# Autodesk Inventor assembly: Ramps 1.4
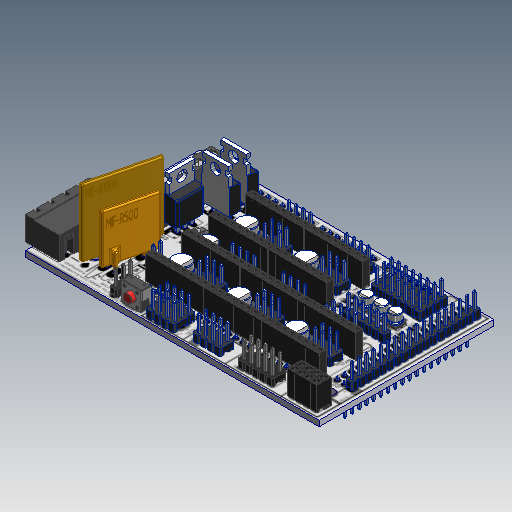
[picture p0: Inventor's stored thumbnail of the model, 512x512]
Saved by Autodesk Inventor 2017 (Build 210142000, 142)
## iProperties
Created: 2012-11-13
Part Number: Ramps 1.4
Document SubType Name: Ensemble
Mass: 53.1508 g
Surface Area: 690.991 cm^2
Volume: 42.1194 cm^3
Density: 1.26191 g/cm^3
Stock Number: 1420-11-20
Sending System: SolidWorks 2013
Preprocessor: SwSTEP 2.0
Title: RAMPS1_4.STEP
## Documents named in this file (24)
- W:\Professionnel\Conception FABLAB\1420-Vauban 3D XL\1420-11 Electronique\1420-11-20 Ramps\1420-11-20 Ramps 1.4.iam
- W:\Professionnel\Conception FABLAB\1420-Vauban 3D XL\1420-11 Electronique\1420-11-20 Ramps\RAMPS1_4.ipt
- W:\Professionnel\Conception FABLAB\1420-Vauban 3D XL\1420-11 Electronique\1420-11-20 Ramps\User Library-POWER MOSFET, NON-SURFACE-MOUNT.ipt
- W:\Professionnel\Conception FABLAB\1420-Vauban 3D XL\1420-11 Electronique\1420-11-20 Ramps\female_header_a-bl254-dg-g08d.ipt
- W:\Professionnel\Conception FABLAB\1420-Vauban 3D XL\1420-11 Electronique\1420-11-20 Ramps\female_header_a-bl254-eg-g08d.ipt
- W:\Professionnel\Conception FABLAB\1420-Vauban 3D XL\1420-11 Electronique\1420-11-20 Ramps\pin_header_aw254-dg-g36d.ipt
- W:\Professionnel\Conception FABLAB\1420-Vauban 3D XL\1420-11 Electronique\1420-11-20 Ramps\pin_header_aw140-eg-g18d.ipt
- W:\Professionnel\Conception FABLAB\1420-Vauban 3D XL\1420-11 Electronique\1420-11-20 Ramps\pin_header_aw140-eg-g08d.ipt
- W:\Professionnel\Conception FABLAB\1420-Vauban 3D XL\1420-11 Electronique\1420-11-20 Ramps\pin_header_aw140-eg-g06d.ipt
- W:\Professionnel\Conception FABLAB\1420-Vauban 3D XL\1420-11 Electronique\1420-11-20 Ramps\pin_header_aw140-eg-g04d.ipt
- W:\Professionnel\Conception FABLAB\1420-Vauban 3D XL\1420-11 Electronique\1420-11-20 Ramps\pin_header_aw254-dg-g06d.ipt
- W:\Professionnel\Conception FABLAB\1420-Vauban 3D XL\1420-11 Electronique\1420-11-20 Ramps\pin_header_aw254-dg-g08d.ipt
- W:\Professionnel\Conception FABLAB\1420-Vauban 3D XL\1420-11 Electronique\1420-11-20 Ramps\pin_header_aw254-dg-g10d.ipt
- W:\Professionnel\Conception FABLAB\1420-Vauban 3D XL\1420-11 Electronique\1420-11-20 Ramps\terminal_blocks_a-tb500-to06.ipt
- W:\Professionnel\Conception FABLAB\1420-Vauban 3D XL\1420-11 Electronique\1420-11-20 Ramps\terminal_blocks_a-tb508-oq04ch.ipt
- W:\Professionnel\Conception FABLAB\1420-Vauban 3D XL\1420-11 Electronique\1420-11-20 Ramps\pin_header_aw140-eg-g02d.ipt
- W:\Professionnel\Conception FABLAB\1420-Vauban 3D XL\1420-11 Electronique\1420-11-20 Ramps\pin_header_aw140-eg-g03d.ipt
- W:\Professionnel\Conception FABLAB\1420-Vauban 3D XL\1420-11 Electronique\1420-11-20 Ramps\User Library-CAPSMD6_3x3_9.iam
- W:\Professionnel\Conception FABLAB\1420-Vauban 3D XL\1420-11 Electronique\1420-11-20 Ramps\User Library-CAPSMD4x3_9.iam
- W:\Professionnel\Conception FABLAB\1420-Vauban 3D XL\1420-11 Electronique\1420-11-20 Ramps\User Library-APA3010GCCK_GREEN.ipt
- W:\Professionnel\Conception FABLAB\1420-Vauban 3D XL\1420-11 Electronique\1420-11-20 Ramps\User Library-APA3010GCCK_RED.ipt
- W:\Professionnel\Conception FABLAB\1420-Vauban 3D XL\1420-11 Electronique\1420-11-20 Ramps\User Library-MF-R1100___ _________.ipt
- W:\Professionnel\Conception FABLAB\1420-Vauban 3D XL\1420-11 Electronique\1420-11-20 Ramps\User Library-MF-R500___ _________.ipt
- W:\Professionnel\Conception FABLAB\1420-Vauban 3D XL\1420-11 Electronique\1420-11-20 Ramps\User Library-SWITCH, TACTILE, RIGHT ANGLE, 12VDC, 50MA, 6_85MM ACTUATOR, WEALTH METAL TC-0244Z.ipt
## Components (62 placed, 62 different names)
1. RAMPS1_4_1 — Placage:1
2. User Library-POWER MOSFET, NON-SURFACE-MOUNT_2
3. female_header_a-bl254-dg-g08d_3
4. female_header_a-bl254-eg-g08d_4
5. female_header_a-bl254-eg-g08d_5
6. female_header_a-bl254-eg-g08d_6
7. female_header_a-bl254-eg-g08d_7
8. female_header_a-bl254-eg-g08d_8
9. female_header_a-bl254-eg-g08d_9
10. female_header_a-bl254-eg-g08d_10
11. female_header_a-bl254-eg-g08d_11
12. female_header_a-bl254-eg-g08d_12
13. female_header_a-bl254-eg-g08d_13
14. pin_header_aw254-dg-g36d_14
15. pin_header_aw140-eg-g18d_15
16. pin_header_aw140-eg-g08d_16
17. pin_header_aw140-eg-g08d_17
18. pin_header_aw140-eg-g08d_18
19. pin_header_aw140-eg-g08d_19
20. pin_header_aw140-eg-g08d_20
21. pin_header_aw140-eg-g06d_21
22. pin_header_aw140-eg-g06d_22
23. pin_header_aw140-eg-g06d_23
24. pin_header_aw140-eg-g06d_24
25. pin_header_aw140-eg-g04d_25
26. pin_header_aw140-eg-g04d_26
27. pin_header_aw140-eg-g04d_27
28. pin_header_aw140-eg-g04d_28
29. pin_header_aw140-eg-g04d_29
30. pin_header_aw254-dg-g06d_30
31. pin_header_aw254-dg-g06d_31
32. pin_header_aw254-dg-g06d_32
33. pin_header_aw254-dg-g06d_33
34. pin_header_aw254-dg-g06d_34
35. pin_header_aw254-dg-g08d_35
36. pin_header_aw254-dg-g08d_36
37. pin_header_aw254-dg-g10d_37
38. pin_header_aw140-eg-g04d_38
39. pin_header_aw140-eg-g06d_39
40. terminal_blocks_a-tb500-to06_40
41. terminal_blocks_a-tb508-oq04ch_41
42. pin_header_aw254-dg-g08d_42
43. pin_header_aw140-eg-g02d_43
44. pin_header_aw140-eg-g03d_44
45. User Library-CAPSMD6_3x3_9_46 [sub-assembly]
46. User Library-CAPSMD6_3x3_9_47 [sub-assembly]
47. User Library-CAPSMD6_3x3_9_48 [sub-assembly]
48. User Library-CAPSMD6_3x3_9_49 [sub-assembly]
49. User Library-CAPSMD6_3x3_9_50 [sub-assembly]
50. User Library-CAPSMD6_3x3_9_51 [sub-assembly]
51. User Library-CAPSMD4x3_9_52 [sub-assembly]
52. User Library-CAPSMD4x3_9_53 [sub-assembly]
53. User Library-CAPSMD4x3_9_54 [sub-assembly]
54. User Library-APA3010GCCK_GREEN_55
55. User Library-APA3010GCCK_RED_56
56. User Library-APA3010GCCK_RED_57
57. User Library-MF-R1100___ __________58
58. User Library-MF-R500___ __________59 — Placage:1
59. User Library-SWITCH, TACTILE, RIGHT ANGLE, 12VDC, 50MA, 6_85MM ACTUATOR, WEALTH METAL TC-0244Z_60
60. User Library-APA3010GCCK_RED_61
61. User Library-POWER MOSFET, NON-SURFACE-MOUNT_62
62. User Library-POWER MOSFET, NON-SURFACE-MOUNT_63
## Relationships (1: Mate 1)
- Placage:1 [Mate]: RAMPS1_4_1 ↔ User Library-MF-R500___ __________59
